# Autodesk Inventor assembly: Overhead Bar
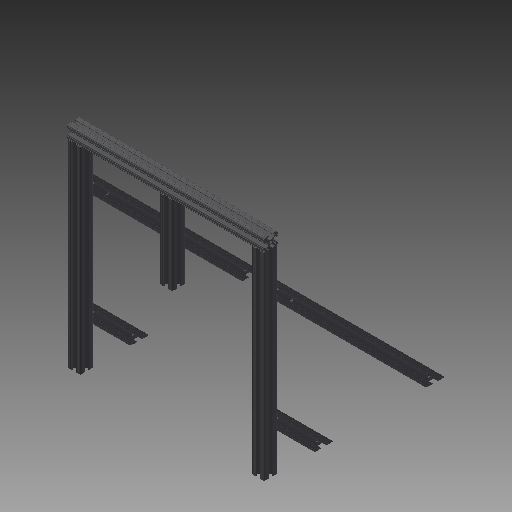
[picture p0: Inventor's stored thumbnail of the model, 512x512]
Saved by Autodesk Inventor 2017 SP1 (Build 210196100, 196)
## iProperties
Created: 2016-04-02
Part Number: Overhead Bar
Document SubType Name: Assembly
Designer: hwasserb
Author: hwasserb
## Documents named in this file (6)
- C:\Users\Haden\Desktop\Charlie-CAD-Model\Robot Model\Overhead Bar\Overhead Bar.iam
- C:\Users\Haden\Desktop\Charlie-CAD-Model\Robot Model\Overhead Bar\Large Angled.ipt
- C:\Users\Haden\Desktop\Charlie-CAD-Model\Robot Model\Overhead Bar\Middle.ipt
- C:\Users\Haden\Desktop\Charlie-CAD-Model\Robot Model\Overhead Bar\Small Angled.ipt
- C:\Users\Haden\Desktop\Charlie-CAD-Model\Robot Model\Overhead Bar\Top.ipt
- C:\Users\Haden\Desktop\Charlie-CAD-Model\Robot Model\Overhead Bar\Vertical.ipt
## Components (8 placed, 5 different names)
1. Large Angled:1 — Mate:11, Flush:15, Flush:16
2. Large Angled:2 — Mate:5, Flush:3, Flush:4
3. Middle:1 — Mate:9, Flush:14, Mate:10
4. Small Angled:1 — Mate:8, Flush:12, Flush:13
5. Small Angled:2 — Mate:6, Flush:8, Flush:9
6. Top:1 — Mate:1, Flush:1, Mate:2, Flush:2, Mate:3, Mate:4, Mate:9, Flush:14, Mate:10
7. Vertical:1 — Mate:1, Flush:1, Mate:3, Mate:8, Flush:12, Flush:13, Mate:11, Flush:15, Flush:16
8. Vertical:2 — Mate:2, Flush:2, Mate:4, Mate:5, Flush:3, Flush:4, Mate:6, Flush:8, Flush:9
## Relationships (21: Flush 11, Mate 10)
- Mate:1: Top:1 ↔ Vertical:1
- Flush:1: Top:1 ↔ Vertical:1
- Mate:2: Top:1 ↔ Vertical:2
- Flush:2: Top:1 ↔ Vertical:2
- Mate:3: Top:1 ↔ Vertical:1
- Mate:4: Top:1 ↔ Vertical:2
- Mate:5: Large Angled:2 ↔ Vertical:2
- Flush:3: Large Angled:2 ↔ Vertical:2
- Flush:4: Large Angled:2 ↔ Vertical:2
- Mate:6: Small Angled:2 ↔ Vertical:2
- Flush:8: Small Angled:2 ↔ Vertical:2
- Flush:9: Small Angled:2 ↔ Vertical:2
- Mate:8: Small Angled:1 ↔ Vertical:1
- Flush:12: Small Angled:1 ↔ Vertical:1
- Flush:13: Small Angled:1 ↔ Vertical:1
- Mate:9: Middle:1 ↔ Top:1
- Flush:14: Middle:1 ↔ Top:1
- Mate:10: Middle:1 ↔ Top:1
- Mate:11: Large Angled:1 ↔ Vertical:1
- Flush:15: Large Angled:1 ↔ Vertical:1
- Flush:16: Large Angled:1 ↔ Vertical:1
